# Autodesk Inventor assembly: 1310164 DHRS-32-A---(0)
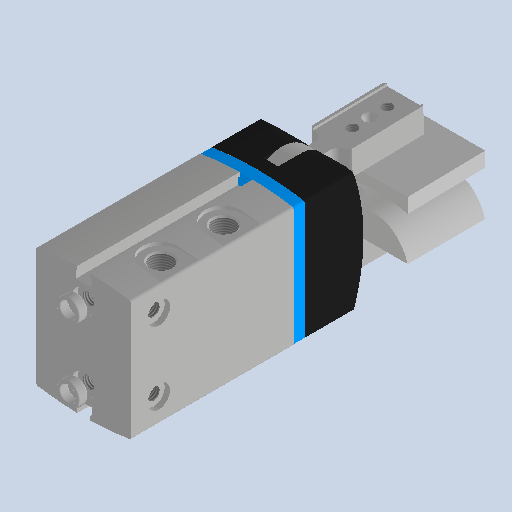
[picture p0: Inventor's stored thumbnail of the model, 512x512]
Saved by Autodesk Inventor 2025.2 (Build 292293000, 293)
## iProperties
Category: PARTsolutions
Company: FESTO
Created: 2025-06-16
Part Number: 1310164 DHRS-32-A---(0)
Catalog Web Link: www.cadenas.de
Description: DHRS-Radial gripper
Vendor: FESTO
Document SubType Name: Assembly
Designer: psAdmin
Manufacturer: FESTO
Mass: 480 g
Surface Area: 329.407 cm^2
Volume: 177.381 cm^3
Density: 2.70604 g/cm^3
PSOL_IDENT_0: {ATYP=ASSISTANT},{DATA=script=$CADENAS_DATA/23d-libs/festo/webfesto.vbb&M_FAMILY=DHRS&M_GROUP=01&M_P
PSOL_IDENT_1: ARTNO=1310164&IDCODE1=DHRS-32-A&IDCODE2=&customer_number_cns=&MATES=1&LOD=HI&LOCKERP=0&SINGLEPART=1}
NB: 1310164 DHRS-32-A---(0)
NN: DHRS
NT: Radial gripper
NBSYN: $TNR. $TYP.---($ROT.)
LINA: 1310164 DHRS-32-A
CATALOG: Festo
TNR: 1310164
TYP: DHRS-32-A
ROT: 0
B1: 38
B2: 0
B3: 11
B4: 16
B5: 14
D1: 4
D2: 5.1
D3: 9
D4: 15
D5: M5
D6: M6
D7: 9
D8: 6.4
EE: G1/8
H1: 128.5
H2: 96.2
H3: 65
H4: 103.5
H5: 29.5
H6: 32
H7: 14
H8: 7
H9: 14
H10: 11
H11: 20
H12: 25
H13: 15
L1: 51
L2: 29
L3: 25.8
L4: 24.8
L5: 8
L6: 1
L7: 10
T1: 2.1
T2: 12.9
T3: 6.5
T4: 24.044
T5: 1.9
W1: 90
W2: 2
CNSMASSEXACT: 0.48
GTIN: 4052568229610
SUPPLIER: FESTO
ARTICLENO: 1310164 DHRS-32-A---(0)
BOMINFO: 1310164 DHRS-32-A
CREATOR: CADENAS GmbH
Title: 1310164 DHRS-32-A
Author: Cadenas PARTsolutions
Comments: Radial gripper
## Documents named in this file (6)
- C:\Users\tino\Documents_VM\Konstruieren_CAD\Useless Box\Kaufteile\DHRS-32-A - Kopie\AIS2024\1310164 DHRS-32-A---(0).iam
- C:\Users\tino\Documents_VM\Konstruieren_CAD\Useless Box\Kaufteile\DHRS-32-A - Kopie\AIS2024\1310164 DHRS-32-A---(Geh).ipt
- C:\Users\tino\Documents_VM\Konstruieren_CAD\Useless Box\Kaufteile\DHRS-32-A - Kopie\AIS2024\1310164 DHRS-32-A---(Griff).ipt
- C:\Users\tino\Documents_VM\Konstruieren_CAD\Useless Box\Kaufteile\DHRS-32-A - Kopie\AIS2024\8137184 ZBH-9-B.ipt
- C:\Users\tino\Documents_VM\Konstruieren_CAD\Useless Box\Eigene Bauteile\ER_Backe_Links_neu.ipt
- C:\Users\tino\Documents_VM\Konstruieren_CAD\Useless Box\Eigene Bauteile\ER_Backe_Rechts_neu.ipt
## Components (7 placed, 5 different names)
1. 1310164 DHRS-32-A---(Geh):1 — TO_JAW_L_XY@1 <-> GRIFF_XY@2, TO_JAW_L_Z@1 <-> GRIFF_Z@2, TO_JAW_L_YZ@1 <-> GRIFF_YZ@2, TO_JAW_R_XY@1 <-> GRIFF_XY@3, TO_JAW_R_Z@1 <-> GRIFF_Z@3, TO_JAW_R_YZ@1 <-> GRIFF_YZ@3, TO_ZBH_1_Z@1 <-> insert_Z@4, TO_ZBH_1_YZ@1 <-> insert_YZ@4, TO_ZBH_2_Z@1 <-> insert_Z@5, TO_ZBH_2_YZ@1 <-> insert_YZ@5
2. 1310164 DHRS-32-A---(Griff):1 — TO_JAW_L_XY@1 <-> GRIFF_XY@2, TO_JAW_L_Z@1 <-> GRIFF_Z@2, TO_JAW_L_YZ@1 <-> GRIFF_YZ@2, Passend:6, Passend:7, Passend:8
3. 1310164 DHRS-32-A---(Griff):2 — TO_JAW_R_XY@1 <-> GRIFF_XY@3, TO_JAW_R_Z@1 <-> GRIFF_Z@3, TO_JAW_R_YZ@1 <-> GRIFF_YZ@3, Passend:9, Passend:10, Passend:11
4. 8137184 ZBH-9-B:1 — TO_ZBH_1_Z@1 <-> insert_Z@4, TO_ZBH_1_YZ@1 <-> insert_YZ@4
5. 8137184 ZBH-9-B:2 — TO_ZBH_2_Z@1 <-> insert_Z@5, TO_ZBH_2_YZ@1 <-> insert_YZ@5
6. ER_Backe_Links_neu:1 — Passend:6, Passend:7, Passend:8
7. ER_Backe_Rechts_neu:1 — Passend:9, Passend:10, Passend:11
## Relationships (16: Mate 11, Angle 4, Flush 1)
- TO_JAW_L_XY@1 <-> GRIFF_XY@2 [Flush]: 1310164 DHRS-32-A---(Geh):1 ↔ 1310164 DHRS-32-A---(Griff):1
- TO_JAW_L_Z@1 <-> GRIFF_Z@2 [Mate]: 1310164 DHRS-32-A---(Geh):1 ↔ 1310164 DHRS-32-A---(Griff):1
- TO_JAW_L_YZ@1 <-> GRIFF_YZ@2 [Angle] (-2 deg): 1310164 DHRS-32-A---(Geh):1 ↔ 1310164 DHRS-32-A---(Griff):1
- TO_JAW_R_XY@1 <-> GRIFF_XY@3 [Mate]: 1310164 DHRS-32-A---(Geh):1 ↔ 1310164 DHRS-32-A---(Griff):2
- TO_JAW_R_Z@1 <-> GRIFF_Z@3 [Mate]: 1310164 DHRS-32-A---(Geh):1 ↔ 1310164 DHRS-32-A---(Griff):2
- TO_JAW_R_YZ@1 <-> GRIFF_YZ@3 [Angle] (182 deg): 1310164 DHRS-32-A---(Geh):1 ↔ 1310164 DHRS-32-A---(Griff):2
- TO_ZBH_1_Z@1 <-> insert_Z@4 [Mate]: 1310164 DHRS-32-A---(Geh):1 ↔ 8137184 ZBH-9-B:1
- TO_ZBH_1_YZ@1 <-> insert_YZ@4 [Angle] (0 deg): 1310164 DHRS-32-A---(Geh):1 ↔ 8137184 ZBH-9-B:1
- TO_ZBH_2_Z@1 <-> insert_Z@5 [Mate]: 1310164 DHRS-32-A---(Geh):1 ↔ 8137184 ZBH-9-B:2
- TO_ZBH_2_YZ@1 <-> insert_YZ@5 [Angle] (0 deg): 1310164 DHRS-32-A---(Geh):1 ↔ 8137184 ZBH-9-B:2
- Passend:6 [Mate]: 1310164 DHRS-32-A---(Griff):1 ↔ ER_Backe_Links_neu:1
- Passend:7 [Mate]: 1310164 DHRS-32-A---(Griff):1 ↔ ER_Backe_Links_neu:1
- Passend:8 [Mate]: 1310164 DHRS-32-A---(Griff):1 ↔ ER_Backe_Links_neu:1
- Passend:9 [Mate]: 1310164 DHRS-32-A---(Griff):2 ↔ ER_Backe_Rechts_neu:1
- Passend:10 [Mate]: 1310164 DHRS-32-A---(Griff):2 ↔ ER_Backe_Rechts_neu:1
- Passend:11 [Mate]: 1310164 DHRS-32-A---(Griff):2 ↔ ER_Backe_Rechts_neu:1
